# Autodesk Inventor assembly: square_assem
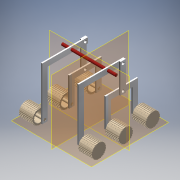
[picture p0: Inventor's stored thumbnail of the model, 180x180]
Saved by Autodesk Inventor 2018.1 (Build 221171000, 171)
## iProperties
Created: 2017-10-26
Part Number: square_assem
Material: 一般
Document SubType Name: Assembly
Designer: Kakeru Yamashita
Author: Kakeru Yamashita
## Documents named in this file (10)
- C:\Users\Kakeru Yamashita\Documents\Inventor\forest_cad-master\Rocker_bogie_sim\square_assem.iam
- C:\Users\Kakeru Yamashita\Documents\Inventor\forest_cad-master\Rocker_bogie_sim\tire.ipt
- C:\Users\Kakeru Yamashita\Documents\Inventor\forest_cad-master\Rocker_bogie_sim\bogie_square.ipt
- C:\Users\Kakeru Yamashita\Documents\Inventor\forest_cad-master\Rocker_bogie_sim\rocker.ipt
- C:\Users\Kakeru Yamashita\Documents\Inventor\forest_cad-master\Rocker_bogie_sim\rocker_bogie_plate.ipt
- C:\Users\Kakeru Yamashita\Documents\Inventor\forest_cad-master\Rocker_bogie_sim\sim_shaft.ipt
- C:\Users\Kakeru Yamashita\Documents\Inventor\forest_cad-master\Rocker_bogie_sim\tire_MIR.ipt
- C:\Users\Kakeru Yamashita\Documents\Inventor\forest_cad-master\Rocker_bogie_sim\bogie_square_MIR.ipt
- C:\Users\Kakeru Yamashita\Documents\Inventor\forest_cad-master\Rocker_bogie_sim\rocker_MIR.ipt
- C:\Users\Kakeru Yamashita\Documents\Inventor\forest_cad-master\Rocker_bogie_sim\rocker_bogie_plate_MIR.ipt
## Components (13 placed, 9 different names)
1. tire:1 — フラッシュ:1, メイト:2, フラッシュ:2
2. tire:2 — フラッシュ:1, メイト:1, フラッシュ:5
3. bogie_square:1 — メイト:1, メイト:2, フラッシュ:2, メイト:4, メイト:7, フラッシュ:11
4. rocker:1 — メイト:3, フラッシュ:6, メイト:5, メイト:6, フラッシュ:7, メイト:8, フラッシュ:9, フラッシュ:10, フラッシュ:12
5. tire:3 — フラッシュ:5, メイト:3, フラッシュ:6
6. rocker_bogie_plate:1 — メイト:4, メイト:5, メイト:6, メイト:7, フラッシュ:7, フラッシュ:11
7. sim_shaft:1 — フラッシュ:8, メイト:8, フラッシュ:9, フラッシュ:21
8. tire_MIR:1 — フラッシュ:13, フラッシュ:14, メイト:9
9. tire_MIR:2 — フラッシュ:13, メイト:10, フラッシュ:18
10. bogie_square_MIR:1 — フラッシュ:14, メイト:9, メイト:10, フラッシュ:19, メイト:12, メイト:15
11. rocker_MIR:1 — フラッシュ:15, フラッシュ:16, フラッシュ:17, メイト:11, フラッシュ:20, メイト:13, メイト:14, フラッシュ:21
12. tire_MIR:3 — フラッシュ:17, メイト:11, フラッシュ:18
13. rocker_bogie_plate_MIR:1 — フラッシュ:19, フラッシュ:20, メイト:12, メイト:13, メイト:14, メイト:15
## Relationships (34: Flush 19, Mate 15)
- フラッシュ:1 [Flush]: tire:1 ↔ tire:2
- メイト:1 [Mate]: tire:2 ↔ bogie_square:1
- メイト:2 [Mate]: tire:1 ↔ bogie_square:1
- フラッシュ:2 [Flush]: tire:1 ↔ bogie_square:1
- フラッシュ:5 [Flush]: tire:2 ↔ tire:3
- メイト:3 [Mate]: rocker:1 ↔ tire:3
- フラッシュ:6 [Flush]: rocker:1 ↔ tire:3
- メイト:4 [Mate]: bogie_square:1 ↔ rocker_bogie_plate:1
- メイト:5 [Mate]: rocker:1 ↔ rocker_bogie_plate:1
- メイト:6 [Mate]: rocker:1 ↔ rocker_bogie_plate:1
- メイト:7 [Mate]: bogie_square:1 ↔ rocker_bogie_plate:1
- フラッシュ:7 [Flush]: rocker:1 ↔ rocker_bogie_plate:1
- フラッシュ:8 [Flush] (100 mm): sim_shaft:1
- メイト:8 [Mate]: rocker:1 ↔ sim_shaft:1
- フラッシュ:9 [Flush] (30 mm): rocker:1 ↔ sim_shaft:1
- フラッシュ:10 [Flush] (110 mm): rocker:1
- フラッシュ:11 [Flush]: bogie_square:1 ↔ rocker_bogie_plate:1
- フラッシュ:12 [Flush] (210 mm): rocker:1
- フラッシュ:13 [Flush]: tire_MIR:1 ↔ tire_MIR:2
- フラッシュ:14 [Flush]: tire_MIR:1 ↔ bogie_square_MIR:1
- メイト:9 [Mate]: tire_MIR:1 ↔ bogie_square_MIR:1
- メイト:10 [Mate]: tire_MIR:2 ↔ bogie_square_MIR:1
- フラッシュ:15 [Flush] (210 mm): rocker_MIR:1
- フラッシュ:16 [Flush] (110 mm): rocker_MIR:1
- フラッシュ:17 [Flush]: rocker_MIR:1 ↔ tire_MIR:3
- メイト:11 [Mate]: rocker_MIR:1 ↔ tire_MIR:3
- フラッシュ:18 [Flush]: tire_MIR:2 ↔ tire_MIR:3
- フラッシュ:19 [Flush]: bogie_square_MIR:1 ↔ rocker_bogie_plate_MIR:1
- フラッシュ:20 [Flush]: rocker_MIR:1 ↔ rocker_bogie_plate_MIR:1
- メイト:12 [Mate]: bogie_square_MIR:1 ↔ rocker_bogie_plate_MIR:1
- メイト:13 [Mate]: rocker_MIR:1 ↔ rocker_bogie_plate_MIR:1
- メイト:14 [Mate]: rocker_MIR:1 ↔ rocker_bogie_plate_MIR:1
- メイト:15 [Mate]: bogie_square_MIR:1 ↔ rocker_bogie_plate_MIR:1
- フラッシュ:21 [Flush] (30 mm): sim_shaft:1 ↔ rocker_MIR:1
